# Autodesk Inventor assembly: Gripper
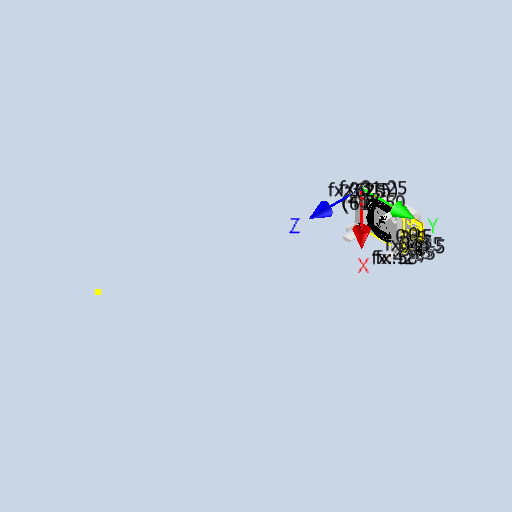
[picture p0: Inventor's stored thumbnail of the model, 512x512]
Saved by Autodesk Inventor 2024 (Build 280153000, 153)
## iProperties
Created: 2024-03-27
Part Number: Gripper
Document SubType Name: Assembly
Designer: jens1
Author: jens1
## Documents named in this file (6)
- C:\Users\jens1\Documents\GitHub\Robotteknologi-2.-semester\3D modeller\Gripper\Gripper.iam
- C:\Users\jens1\Documents\GitHub\Robotteknologi-2.-semester\3D modeller\UR5 gripper mount.ipt
- C:\Users\jens1\Documents\GitHub\Robotteknologi-2.-semester\3D modeller\Gripper\Fake Fuses.ipt
- C:\Users\jens1\Documents\GitHub\Robotteknologi-2.-semester\3D modeller\Gripper\Top bot holder.ipt
- C:\Users\jens1\Documents\GitHub\Robotteknologi-2.-semester\3D modeller\Gripper\Fuse holder V2.ipt
- C:\Users\jens1\Documents\GitHub\Robotteknologi-2.-semester\3D modeller\Gripper\Top bot holder med bund.ipt
## Components (5 placed, 5 different names)
1. UR5 gripper mount:1 — Mate:7, Flush:14, Flush:15, Mate:9, Mate:10, Mate:11, Mate:12, Flush:16, Mate:13, Mate:14, Mate:15, Mate:16
2. Fake Fuses:1 — Flush:15, Mate:11, Mate:12
3. Top bot holder:1 — Mate:7, Flush:16, Mate:13
4. Fuse holder V2:1 — Flush:14, Mate:9, Mate:10
5. Top bot holder med bund:1 — Mate:14, Mate:15, Mate:16
## Relationships (12: Mate 9, Flush 3)
- Mate:7: UR5 gripper mount:1 ↔ Top bot holder:1
- Flush:14: UR5 gripper mount:1 ↔ Fuse holder V2:1
- Flush:15: UR5 gripper mount:1 ↔ Fake Fuses:1
- Mate:9: UR5 gripper mount:1 ↔ Fuse holder V2:1
- Mate:10: UR5 gripper mount:1 ↔ Fuse holder V2:1
- Mate:11: UR5 gripper mount:1 ↔ Fake Fuses:1
- Mate:12: UR5 gripper mount:1 ↔ Fake Fuses:1
- Flush:16 (2.5 mm): UR5 gripper mount:1 ↔ Top bot holder:1
- Mate:13: UR5 gripper mount:1 ↔ Top bot holder:1
- Mate:14: UR5 gripper mount:1 ↔ Top bot holder med bund:1
- Mate:15: UR5 gripper mount:1 ↔ Top bot holder med bund:1
- Mate:16: UR5 gripper mount:1 ↔ Top bot holder med bund:1
